# Autodesk Inventor assembly: steam cylinder 1
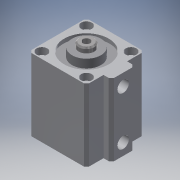
[picture p0: Inventor's stored thumbnail of the model, 180x180]
Saved by Autodesk Inventor 2016 (Build 200138000, 138)
## iProperties
Created: 2017-06-14
Part Number: steam cylinder 1
Document SubType Name: Assembly
Designer: RMcComber
Author: RMcComber
## Documents named in this file (4)
- C:\Users\zimirken\Documents\Steam Engines\two cylinder shaft drive 2\steam cylinder 1.iam
- C:\Users\zimirken\Documents\Steam Engines\two cylinder shaft drive 2\cylinder.ipt
- C:\Users\zimirken\Documents\Steam Engines\two cylinder shaft drive 2\piston.ipt
- C:\Users\zimirken\Documents\Steam Engines\two cylinder shaft drive 2\cylinder cap.ipt
## Components (3 placed, 3 different names)
1. cylinder:1 — Mate:1, Mate:2, Flush:2, Mate:3
2. piston:1 — Mate:1, Mate:3
3. cylinder cap:1 — Mate:2, Flush:2
## Relationships (4: Mate 3, Flush 1)
- Mate:1: cylinder:1 ↔ piston:1
- Mate:2: cylinder:1 ↔ cylinder cap:1
- Flush:2 (-3 mm): cylinder:1 ↔ cylinder cap:1
- Mate:3: cylinder:1 ↔ piston:1
